# Autodesk Inventor assembly: СборОчка
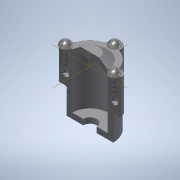
[picture p0: Inventor's stored thumbnail of the model, 180x180]
Saved by Autodesk Inventor 2021 (Build 250183000, 183)
## iProperties
Created: 2020-05-07
Part Number: СборОчка
Material: Типовые
Document SubType Name: Assembly
Designer: 2000
Mass: 415.176 g
Surface Area: 773.527 cm^2
Volume: 291.385 cm^3
Density: 1.42483 g/cm^3
Author: 2000
## Documents named in this file (4)
- C:\Users\2000\Desktop\СборОчка.iam
- C:\Users\2000\Desktop\Деталь1.ipt
- C:\Users\2000\Desktop\Деталь2.ipt
- C:\Users\2000\Documents\Inventor\Content Center Files\R2021\ru-RU\Screw A GOST 17473-80\Винт A.M12-6gx30 ГОСТ 17473-80.ipt
## Components (6 placed, 3 different names)
1. Деталь1:1 — С поворотом:1
2. Деталь2:1 — С поворотом:1
3. Винт A ГОСТ 17473-80 M12-6gx30:1
4. Винт A ГОСТ 17473-80 M12-6gx30:2
5. Винт A ГОСТ 17473-80 M12-6gx30:3
6. Винт A ГОСТ 17473-80 M12-6gx30:4
## Relationships (5: Insert 4, RevoluteJoint 1)
- С поворотом:1 [RevoluteJoint]: Деталь1:1 ↔ Деталь2:1
- [Insert]: Деталь2:1 ↔ Винт A ГОСТ 17473-80 M12-6gx30:1
- [Insert]: Деталь2:1 ↔ Винт A ГОСТ 17473-80 M12-6gx30:2
- [Insert]: Деталь2:1 ↔ Винт A ГОСТ 17473-80 M12-6gx30:3
- [Insert]: Деталь2:1 ↔ Винт A ГОСТ 17473-80 M12-6gx30:4
